# Autodesk Inventor assembly: Assembly Rack_Submission
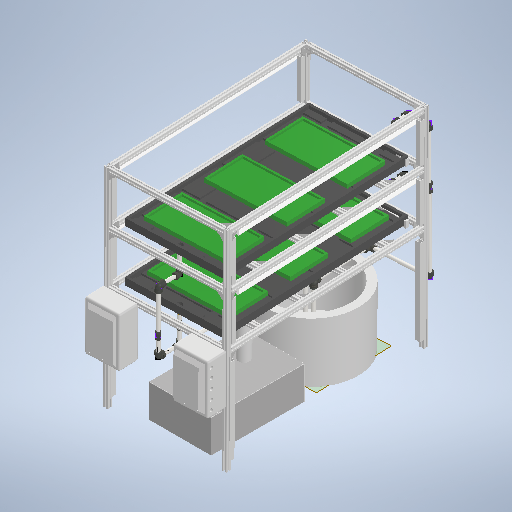
[picture p0: Inventor's stored thumbnail of the model, 512x512]
Saved by Autodesk Inventor 2025 (Build 290162000, 162)
## iProperties
Created: 2024-07-31
Part Number: Assembly Rack_Submission
Document SubType Name: Assembly
Designer: Isaac
Author: Isaac
## Documents named in this file (16)
- C:\Users\User\OneDrive\Documents\FYP\Inventor_Designs\Submission_1\Assembly Rack_Submission.iam
- C:\Users\User\OneDrive\Documents\FYP\Inventor_Designs\Submission_1\Metal_Profile 70cm.ipt
- C:\Users\User\OneDrive\Documents\FYP\Inventor_Designs\Submission_1\Light tube 118.4cm.ipt
- C:\Users\User\OneDrive\Documents\FYP\Inventor_Designs\Submission_1\flood tray.ipt
- C:\Users\User\OneDrive\Documents\FYP\Inventor_Designs\Platform\Potting Tray.ipt
- C:\Users\User\OneDrive\Documents\FYP\Inventor_Designs\Submission_1\Metal Profile 129 cm.ipt
- C:\Users\User\OneDrive\Documents\FYP\Inventor_Designs\Submission_1\Metal Profile 134 cm.ipt
- C:\Users\User\OneDrive\Documents\FYP\Inventor_Designs\L Bracket\L Angle Bracket 30x30.ipt
- C:\Users\User\OneDrive\Documents\FYP\Inventor_Designs\Submission_1\Tub.ipt
- C:\Users\User\OneDrive\Documents\FYP\Inventor_Designs\Submission_1\Water pump.ipt
- C:\Users\User\OneDrive\Documents\FYP\Inventor_Designs\Submission_1\wire box and cover.iam
- C:\Users\User\OneDrive\Documents\FYP\Inventor_Designs\Submission_1\25 cm trunk.ipt
- C:\Users\User\OneDrive\Documents\FYP\Inventor_Designs\Submission_1\55 cm trunk.ipt
- C:\Users\User\OneDrive\Documents\FYP\Inventor_Designs\Submission_1\Part245.ipt
- C:\Users\User\OneDrive\Documents\FYP\Inventor_Designs\Submission_1\Assembly Rack_Submission\AIP\Tube and Pipe\Run03\Assembly Rack_Submission.Tube and Pipe Runs.iam
- C:\Users\User\OneDrive\Documents\FYP\Inventor_Designs\Submission_1\Part18.ipt
## Components (108 placed, 15 different names)
1. Metal_Profile 70cm:1
2. Metal_Profile 70cm:2
3. Metal_Profile 70cm:3
4. Metal_Profile 70cm:4
5. Metal_Profile 70cm:5
6. Metal_Profile 70cm:6
7. Light tube 118.4cm:1
8. Light tube 118.4cm:2
9. Light tube 118.4cm:3
10. Light tube 118.4cm:4
11. flood tray:1 — Mate:196, Mate:198
12. Potting Tray:1
13. Potting Tray:2
14. Potting Tray:3
15. Potting Tray:4
16. Potting Tray:5
17. Potting Tray:6
18. Metal_Profile 70cm:7
19. Metal_Profile 70cm:8
20. flood tray:2
21. Metal Profile 129 cm:1
22. Metal Profile 129 cm:2
23. Metal Profile 129 cm:3
24. Metal Profile 129 cm:4
25. Metal Profile 134 cm:1
26. Metal Profile 134 cm:2 — Flush:117
27. Metal Profile 134 cm:3
28. Metal Profile 134 cm:4
29. Metal Profile 129 cm:5
30. Metal Profile 129 cm:6
31. Metal_Profile 70cm:9
32. Metal_Profile 70cm:10
33. Metal_Profile 70cm:11
34. Metal_Profile 70cm:12
35. Metal_Profile 70cm:13
36. Metal_Profile 70cm:14
37. L Angle Bracket 30x30:1
38. L Angle Bracket 30x30:2
39. L Angle Bracket 30x30:3
40. L Angle Bracket 30x30:4
41. L Angle Bracket 30x30:5
42. L Angle Bracket 30x30:6
43. L Angle Bracket 30x30:7
44. L Angle Bracket 30x30:8
45. L Angle Bracket 30x30:9
46. L Angle Bracket 30x30:10
47. L Angle Bracket 30x30:11
48. L Angle Bracket 30x30:12
49. L Angle Bracket 30x30:13
50. L Angle Bracket 30x30:14
51. L Angle Bracket 30x30:15
52. L Angle Bracket 30x30:16
53. L Angle Bracket 30x30:17
54. L Angle Bracket 30x30:18
55. L Angle Bracket 30x30:19
56. L Angle Bracket 30x30:20
57. L Angle Bracket 30x30:21
58. L Angle Bracket 30x30:22
59. L Angle Bracket 30x30:23
60. L Angle Bracket 30x30:24
61. L Angle Bracket 30x30:25
62. L Angle Bracket 30x30:26
63. L Angle Bracket 30x30:27
64. L Angle Bracket 30x30:28
65. L Angle Bracket 30x30:29
66. L Angle Bracket 30x30:30
67. L Angle Bracket 30x30:31
68. L Angle Bracket 30x30:32
69. L Angle Bracket 30x30:33
70. L Angle Bracket 30x30:34
71. L Angle Bracket 30x30:35
72. L Angle Bracket 30x30:36
73. L Angle Bracket 30x30:37
74. L Angle Bracket 30x30:38
75. L Angle Bracket 30x30:39
76. L Angle Bracket 30x30:40
77. L Angle Bracket 30x30:41
78. L Angle Bracket 30x30:42
79. L Angle Bracket 30x30:43
80. L Angle Bracket 30x30:44
81. L Angle Bracket 30x30:45
82. L Angle Bracket 30x30:46
83. L Angle Bracket 30x30:47
84. L Angle Bracket 30x30:48
85. L Angle Bracket 30x30:49
86. L Angle Bracket 30x30:50
87. L Angle Bracket 30x30:51
88. L Angle Bracket 30x30:52
89. Tub:1 — Mate:198, Flush:117
90. Tube & Pipe Runs [sub-assembly]
91. Water pump:1 — Mate:196, Mate:197
92. wire box and cover:1 [sub-assembly]
93. wire box and cover:2 [sub-assembly]
94. 25 cm trunk:1
95. 25 cm trunk:2
96. 25 cm trunk:3
97. 25 cm trunk:4
98. 25 cm trunk:5
99. 25 cm trunk:6
100. 25 cm trunk:7
101. 25 cm trunk:8
102. 55 cm trunk:1
103. 55 cm trunk:2
104. 55 cm trunk:3
105. 55 cm trunk:4 — Mate:197
106. Part245:1
107. Part18:3
108. Part18:4
## Relationships (315: Mate 198, Flush 117)
- [Flush] (60 mm): Metal_Profile 70cm:3 ↔ flood tray:1
- [Mate]: flood tray:1 ↔ Potting Tray:3
- [Mate]: flood tray:1 ↔ Potting Tray:1
- [Mate]: flood tray:1 ↔ Potting Tray:2
- [Mate] (30 mm): flood tray:1 ↔ Potting Tray:3
- [Mate] (50 mm): flood tray:1 ↔ Potting Tray:3
- [Mate] (30 mm): flood tray:1 ↔ Potting Tray:1
- [Mate] (150 mm): Potting Tray:1 ↔ Potting Tray:3
- [Mate] (30 mm): flood tray:1 ↔ Potting Tray:2
- [Mate] (150 mm): Potting Tray:1 ↔ Potting Tray:2
- [Mate] (150 mm): Potting Tray:4 ↔ Potting Tray:5
- [Mate] (150 mm): Potting Tray:5 ↔ Potting Tray:6
- [Mate]: Metal_Profile 70cm:8 ↔ flood tray:2
- [Flush]: flood tray:1 ↔ flood tray:2
- [Flush]: flood tray:1 ↔ flood tray:2
- [Flush]: Metal_Profile 70cm:5 ↔ Metal Profile 129 cm:3
- [Mate]: Metal_Profile 70cm:5 ↔ Metal Profile 129 cm:1
- [Flush]: Metal_Profile 70cm:5 ↔ Metal Profile 129 cm:1
- [Mate]: Metal_Profile 70cm:5 ↔ Metal Profile 134 cm:2
- [Flush]: Metal_Profile 70cm:5 ↔ Metal Profile 134 cm:2
- [Flush]: Metal Profile 129 cm:1 ↔ Metal Profile 134 cm:2
- [Flush]: Metal_Profile 70cm:5 ↔ Metal Profile 134 cm:1
- [Mate]: Metal_Profile 70cm:5 ↔ Metal Profile 134 cm:1
- [Flush]: Metal_Profile 70cm:5 ↔ Metal Profile 134 cm:1
- [Flush]: Metal_Profile 70cm:5 ↔ Metal Profile 134 cm:1
- [Flush]: Metal_Profile 70cm:5 ↔ Metal Profile 129 cm:3
- [Flush]: Metal Profile 129 cm:3 ↔ Metal Profile 134 cm:1
- [Mate]: Metal Profile 129 cm:3 ↔ Metal Profile 134 cm:1
- [Flush]: Metal Profile 129 cm:1 ↔ Metal Profile 134 cm:4
- [Mate]: Metal_Profile 70cm:6 ↔ Metal Profile 134 cm:4
- [Mate]: Metal Profile 129 cm:1 ↔ Metal Profile 134 cm:4
- [Flush]: Metal Profile 129 cm:3 ↔ Metal Profile 134 cm:3
- [Mate]: Metal Profile 129 cm:3 ↔ Metal Profile 134 cm:3
- [Mate]: Metal_Profile 70cm:6 ↔ Metal Profile 134 cm:3
- [Flush]: Metal_Profile 70cm:1 ↔ Metal Profile 129 cm:6
- [Mate]: Metal Profile 134 cm:1 ↔ Metal Profile 129 cm:6
- [Flush]: Metal Profile 134 cm:1 ↔ Metal Profile 129 cm:6
- [Mate]: Metal Profile 129 cm:4 ↔ Metal Profile 134 cm:2
- [Flush]: Metal Profile 129 cm:4 ↔ Metal Profile 134 cm:2
- [Mate]: Metal Profile 134 cm:1 ↔ Metal Profile 129 cm:5
- [Flush]: Metal Profile 134 cm:1 ↔ Metal Profile 129 cm:5
- [Mate]: Metal Profile 129 cm:2 ↔ Metal Profile 134 cm:2
- [Flush]: Metal Profile 129 cm:2 ↔ Metal Profile 134 cm:2
- [Flush]: Metal_Profile 70cm:5 ↔ Metal Profile 134 cm:2
- [Mate]: Metal_Profile 70cm:6 ↔ Metal Profile 129 cm:1
- [Flush]: Metal Profile 129 cm:3 ↔ Metal Profile 134 cm:3
- [Flush]: Metal_Profile 70cm:6 ↔ Metal Profile 134 cm:3
- [Flush] (330 mm): Metal Profile 129 cm:3 ↔ Metal Profile 129 cm:5
- [Flush] (330 mm): Metal Profile 129 cm:5 ↔ Metal Profile 129 cm:6
- [Flush] (330 mm): Metal Profile 129 cm:2 ↔ Metal Profile 129 cm:4
- [Flush]: Metal_Profile 70cm:1 ↔ Metal Profile 134 cm:2
- [Mate]: Metal_Profile 70cm:1 ↔ Metal Profile 134 cm:1
- [Flush]: Metal_Profile 70cm:3 ↔ Metal Profile 134 cm:1
- [Mate]: Metal_Profile 70cm:3 ↔ Metal Profile 134 cm:1
- [Flush]: Metal_Profile 70cm:3 ↔ Metal Profile 129 cm:2
- [Flush]: Metal_Profile 70cm:1 ↔ Metal Profile 129 cm:4
- [Flush]: Metal_Profile 70cm:2 ↔ Metal Profile 129 cm:6
- [Flush]: Metal_Profile 70cm:2 ↔ Metal Profile 134 cm:3
- [Mate]: Metal_Profile 70cm:2 ↔ Metal Profile 134 cm:3
- [Flush]: Metal_Profile 70cm:4 ↔ Metal Profile 129 cm:5
- [Flush]: Metal_Profile 70cm:4 ↔ Metal Profile 134 cm:3
- [Mate]: Metal_Profile 70cm:4 ↔ Metal Profile 134 cm:3
- [Flush]: Light tube 118.4cm:3 ↔ Metal Profile 129 cm:3
- [Mate] (50 mm): Light tube 118.4cm:3 ↔ Metal Profile 134 cm:1
- [Mate]: Light tube 118.4cm:3 ↔ Metal Profile 129 cm:3
- [Mate]: Light tube 118.4cm:2 ↔ Metal Profile 129 cm:5
- [Flush]: Light tube 118.4cm:2 ↔ Metal Profile 129 cm:5
- [Mate] (50 mm): Light tube 118.4cm:2 ↔ Metal Profile 134 cm:1
- [Flush]: Light tube 118.4cm:1 ↔ Metal Profile 129 cm:1
- [Mate] (50 mm): Light tube 118.4cm:1 ↔ Metal Profile 134 cm:2
- [Mate]: Light tube 118.4cm:1 ↔ Metal Profile 129 cm:1
- [Mate] (50 mm): Light tube 118.4cm:4 ↔ Metal Profile 134 cm:2
- [Flush]: Light tube 118.4cm:4 ↔ Metal Profile 129 cm:2
- [Mate]: Light tube 118.4cm:4 ↔ Metal Profile 129 cm:2
- [Mate]: Metal_Profile 70cm:7 ↔ Metal Profile 129 cm:6
- [Flush]: Metal_Profile 70cm:7 ↔ Metal Profile 129 cm:6
- [Mate] (200 mm): Metal_Profile 70cm:1 ↔ Metal_Profile 70cm:7
- [Flush]: Metal_Profile 70cm:8 ↔ Metal Profile 129 cm:6
- [Mate]: Metal_Profile 70cm:8 ↔ Metal Profile 129 cm:6
- [Mate] (200 mm): Metal_Profile 70cm:2 ↔ Metal_Profile 70cm:8
- [Mate]: Metal Profile 129 cm:6 ↔ Metal_Profile 70cm:12
- [Flush]: Metal Profile 129 cm:6 ↔ Metal_Profile 70cm:12
- [Mate] (255 mm): Metal_Profile 70cm:7 ↔ Metal_Profile 70cm:12
- [Mate]: Metal Profile 129 cm:6 ↔ Metal_Profile 70cm:11
- [Flush]: Metal Profile 129 cm:6 ↔ Metal_Profile 70cm:11
- [Mate] (255 mm): Metal_Profile 70cm:8 ↔ Metal_Profile 70cm:11
- [Mate]: Metal Profile 129 cm:5 ↔ Metal_Profile 70cm:10
- [Flush]: Metal Profile 129 cm:5 ↔ Metal_Profile 70cm:10
- [Mate] (200 mm): Metal_Profile 70cm:3 ↔ Metal_Profile 70cm:10
- [Mate]: Metal Profile 129 cm:5 ↔ Metal_Profile 70cm:9
- [Flush]: Metal Profile 129 cm:5 ↔ Metal_Profile 70cm:9
- [Mate] (255 mm): Metal_Profile 70cm:9 ↔ Metal_Profile 70cm:10
- [Mate]: Metal Profile 129 cm:5 ↔ Metal_Profile 70cm:14
- [Flush]: Metal Profile 129 cm:5 ↔ Metal_Profile 70cm:14
- [Mate] (200 mm): Metal_Profile 70cm:4 ↔ Metal_Profile 70cm:14
- [Mate]: Metal Profile 129 cm:5 ↔ Metal_Profile 70cm:13
- [Flush]: Metal Profile 129 cm:5 ↔ Metal_Profile 70cm:13
- [Mate] (255 mm): Metal_Profile 70cm:13 ↔ Metal_Profile 70cm:14
- [Mate]: Metal_Profile 70cm:7 ↔ flood tray:2
- [Flush] (75 mm): flood tray:2 ↔ Metal Profile 129 cm:6
- [Mate]: flood tray:1 ↔ Metal_Profile 70cm:9
- [Flush]: Metal Profile 129 cm:1 ↔ L Angle Bracket 30x30:1
- [Mate]: Metal_Profile 70cm:5 ↔ L Angle Bracket 30x30:1
- [Mate]: Metal Profile 129 cm:1 ↔ L Angle Bracket 30x30:1
- [Mate]: Metal Profile 129 cm:1 ↔ L Angle Bracket 30x30:6
- [Flush]: Metal Profile 129 cm:1 ↔ L Angle Bracket 30x30:6
- [Mate]: Metal_Profile 70cm:6 ↔ L Angle Bracket 30x30:6
- [Flush]: Metal Profile 129 cm:2 ↔ L Angle Bracket 30x30:5
- [Mate]: Metal_Profile 70cm:4 ↔ L Angle Bracket 30x30:4
- [Flush]: Metal_Profile 70cm:4 ↔ L Angle Bracket 30x30:4
- [Mate]: Metal Profile 129 cm:2 ↔ L Angle Bracket 30x30:4
- [Mate]: Metal Profile 129 cm:2 ↔ L Angle Bracket 30x30:5
- [Flush]: Metal Profile 129 cm:2 ↔ L Angle Bracket 30x30:5
- [Mate]: Metal_Profile 70cm:14 ↔ L Angle Bracket 30x30:5
- [Flush]: Metal Profile 129 cm:2 ↔ L Angle Bracket 30x30:7
- [Mate]: Metal_Profile 70cm:13 ↔ L Angle Bracket 30x30:2
- [Mate]: Metal Profile 129 cm:2 ↔ L Angle Bracket 30x30:2
- [Flush]: Metal Profile 129 cm:2 ↔ L Angle Bracket 30x30:2
- [Flush]: Metal Profile 129 cm:2 ↔ L Angle Bracket 30x30:7
- [Mate]: Metal_Profile 70cm:9 ↔ L Angle Bracket 30x30:7
- [Mate]: Metal Profile 129 cm:2 ↔ L Angle Bracket 30x30:7
- [Mate]: Metal_Profile 70cm:10 ↔ L Angle Bracket 30x30:3
- [Flush]: Metal_Profile 70cm:10 ↔ L Angle Bracket 30x30:3
- [Mate]: Metal Profile 129 cm:2 ↔ L Angle Bracket 30x30:3
- [Flush]: Metal Profile 129 cm:4 ↔ L Angle Bracket 30x30:10
- [Mate]: Metal Profile 129 cm:4 ↔ L Angle Bracket 30x30:10
- [Mate]: Metal_Profile 70cm:2 ↔ L Angle Bracket 30x30:10
- [Mate]: Metal_Profile 70cm:8 ↔ L Angle Bracket 30x30:12
- [Mate]: Metal Profile 129 cm:4 ↔ L Angle Bracket 30x30:12
- [Flush]: Metal Profile 129 cm:4 ↔ L Angle Bracket 30x30:12
- [Mate]: Metal_Profile 70cm:11 ↔ L Angle Bracket 30x30:8
- [Flush]: Metal_Profile 70cm:11 ↔ L Angle Bracket 30x30:8
- [Mate]: Metal Profile 129 cm:4 ↔ L Angle Bracket 30x30:8
- [Flush]: Metal_Profile 70cm:12 ↔ L Angle Bracket 30x30:11
- [Mate]: Metal Profile 129 cm:4 ↔ L Angle Bracket 30x30:11
- [Mate]: Metal_Profile 70cm:12 ↔ L Angle Bracket 30x30:11
- [Flush]: Metal Profile 129 cm:4 ↔ L Angle Bracket 30x30:11
- [Mate]: Metal_Profile 70cm:7 ↔ L Angle Bracket 30x30:9
- [Flush]: Metal_Profile 70cm:7 ↔ L Angle Bracket 30x30:9
- [Mate]: Metal Profile 129 cm:4 ↔ L Angle Bracket 30x30:9
- [Mate]: Metal_Profile 70cm:3 ↔ L Angle Bracket 30x30:13
- [Mate]: Metal Profile 129 cm:2 ↔ L Angle Bracket 30x30:13
- [Flush]: Metal_Profile 70cm:1 ↔ L Angle Bracket 30x30:14
- [Mate]: Metal_Profile 70cm:1 ↔ L Angle Bracket 30x30:14
- [Flush]: Metal_Profile 70cm:1 ↔ L Angle Bracket 30x30:14
- [Mate]: Metal Profile 129 cm:4 ↔ L Angle Bracket 30x30:14
- [Mate]: Metal_Profile 70cm:5 ↔ L Angle Bracket 30x30:15
- [Flush]: Metal Profile 134 cm:2 ↔ L Angle Bracket 30x30:15
- [Mate]: Metal Profile 134 cm:2 ↔ L Angle Bracket 30x30:15
- [Mate]: Metal_Profile 70cm:3 ↔ L Angle Bracket 30x30:16
- [Flush]: Metal Profile 134 cm:2 ↔ L Angle Bracket 30x30:16
- [Mate]: Metal Profile 134 cm:2 ↔ L Angle Bracket 30x30:16
- [Mate]: Metal_Profile 70cm:1 ↔ L Angle Bracket 30x30:26
- [Flush]: Metal_Profile 70cm:1 ↔ L Angle Bracket 30x30:26
- [Mate]: Metal Profile 134 cm:2 ↔ L Angle Bracket 30x30:26
- [Mate]: Metal_Profile 70cm:6 ↔ L Angle Bracket 30x30:23
- [Flush]: Metal_Profile 70cm:6 ↔ L Angle Bracket 30x30:23
- [Mate]: Metal Profile 134 cm:4 ↔ L Angle Bracket 30x30:23
- [Mate]: Metal_Profile 70cm:4 ↔ L Angle Bracket 30x30:19
- [Flush]: Metal Profile 134 cm:4 ↔ L Angle Bracket 30x30:19
- [Mate]: Metal Profile 134 cm:4 ↔ L Angle Bracket 30x30:19
- [Mate]: Metal_Profile 70cm:2 ↔ L Angle Bracket 30x30:22
- [Flush]: Metal Profile 134 cm:4 ↔ L Angle Bracket 30x30:22
- [Mate]: Metal Profile 134 cm:4 ↔ L Angle Bracket 30x30:22
- [Mate]: Metal_Profile 70cm:5 ↔ L Angle Bracket 30x30:24
- [Flush]: Metal Profile 134 cm:1 ↔ L Angle Bracket 30x30:24
- [Mate]: Metal Profile 134 cm:1 ↔ L Angle Bracket 30x30:24
- [Mate]: Metal_Profile 70cm:3 ↔ L Angle Bracket 30x30:17
- [Flush]: Metal Profile 134 cm:1 ↔ L Angle Bracket 30x30:17
- [Mate]: Metal Profile 134 cm:1 ↔ L Angle Bracket 30x30:17
- [Mate]: Metal_Profile 70cm:1 ↔ L Angle Bracket 30x30:25
- [Flush]: Metal Profile 134 cm:1 ↔ L Angle Bracket 30x30:25
- [Mate]: Metal Profile 134 cm:1 ↔ L Angle Bracket 30x30:25
- [Mate]: Metal Profile 129 cm:3 ↔ L Angle Bracket 30x30:18
- [Flush]: Metal Profile 134 cm:1 ↔ L Angle Bracket 30x30:18
- [Mate]: Metal Profile 134 cm:1 ↔ L Angle Bracket 30x30:18
- [Flush]: Metal Profile 134 cm:1 ↔ L Angle Bracket 30x30:21
- [Mate]: Metal Profile 129 cm:5 ↔ L Angle Bracket 30x30:21
- [Mate]: Metal Profile 134 cm:1 ↔ L Angle Bracket 30x30:21
- [Flush]: Metal Profile 134 cm:1 ↔ L Angle Bracket 30x30:20
- [Mate]: Metal Profile 134 cm:1 ↔ L Angle Bracket 30x30:20
- [Mate]: Metal Profile 129 cm:6 ↔ L Angle Bracket 30x30:20
- [Flush]: Metal Profile 134 cm:3 ↔ L Angle Bracket 30x30:29
- [Mate]: Metal Profile 129 cm:6 ↔ L Angle Bracket 30x30:29
- [Mate]: Metal Profile 134 cm:3 ↔ L Angle Bracket 30x30:29
- [Flush]: Metal Profile 134 cm:3 ↔ L Angle Bracket 30x30:28
- [Mate]: Metal Profile 129 cm:5 ↔ L Angle Bracket 30x30:28
- [Mate]: Metal Profile 134 cm:3 ↔ L Angle Bracket 30x30:28
- [Mate]: Metal Profile 129 cm:3 ↔ L Angle Bracket 30x30:27
- [Flush]: Metal Profile 129 cm:3 ↔ L Angle Bracket 30x30:27
- [Mate]: Metal Profile 134 cm:3 ↔ L Angle Bracket 30x30:27
- [Mate]: Metal Profile 129 cm:4 ↔ L Angle Bracket 30x30:30
- [Flush]: Metal Profile 129 cm:4 ↔ L Angle Bracket 30x30:30
- [Mate]: Metal Profile 134 cm:4 ↔ L Angle Bracket 30x30:30
- [Mate]: Metal Profile 129 cm:2 ↔ L Angle Bracket 30x30:31
- [Flush]: Metal Profile 129 cm:2 ↔ L Angle Bracket 30x30:31
- [Mate]: Metal Profile 134 cm:4 ↔ L Angle Bracket 30x30:31
- [Mate]: Metal Profile 129 cm:1 ↔ L Angle Bracket 30x30:32
- [Flush]: Metal Profile 129 cm:1 ↔ L Angle Bracket 30x30:32
- [Mate]: Metal Profile 134 cm:4 ↔ L Angle Bracket 30x30:32
- [Mate]: Metal Profile 129 cm:1 ↔ L Angle Bracket 30x30:34
- [Mate]: Metal Profile 134 cm:2 ↔ L Angle Bracket 30x30:34
- [Flush]: Metal Profile 129 cm:1 ↔ L Angle Bracket 30x30:34
- [Mate]: Metal Profile 129 cm:2 ↔ L Angle Bracket 30x30:35
- [Mate]: Metal Profile 134 cm:2 ↔ L Angle Bracket 30x30:35
- [Flush]: Metal Profile 129 cm:2 ↔ L Angle Bracket 30x30:35
- [Mate]: Metal Profile 129 cm:4 ↔ L Angle Bracket 30x30:33
- [Mate]: Metal Profile 134 cm:2 ↔ L Angle Bracket 30x30:33
- [Flush]: Metal Profile 129 cm:4 ↔ L Angle Bracket 30x30:33
- [Mate]: Metal_Profile 70cm:6 ↔ L Angle Bracket 30x30:36
- [Flush]: Metal_Profile 70cm:6 ↔ L Angle Bracket 30x30:36
- [Mate]: Metal Profile 134 cm:3 ↔ L Angle Bracket 30x30:36
- [Mate]: Metal_Profile 70cm:4 ↔ L Angle Bracket 30x30:37
- [Mate]: Metal Profile 134 cm:3 ↔ L Angle Bracket 30x30:37
- [Flush]: Metal_Profile 70cm:4 ↔ L Angle Bracket 30x30:37
- [Mate]: Metal_Profile 70cm:2 ↔ L Angle Bracket 30x30:38
- [Flush]: Metal_Profile 70cm:2 ↔ L Angle Bracket 30x30:38
- [Mate]: Metal Profile 134 cm:3 ↔ L Angle Bracket 30x30:38
- [Flush]: Metal_Profile 70cm:5 ↔ L Angle Bracket 30x30:40
- [Mate]: Metal Profile 129 cm:3 ↔ L Angle Bracket 30x30:40
- [Mate]: Metal_Profile 70cm:5 ↔ L Angle Bracket 30x30:40
- [Flush]: Metal_Profile 70cm:5 ↔ L Angle Bracket 30x30:40
- [Flush]: Metal_Profile 70cm:3 ↔ L Angle Bracket 30x30:39
- [Mate]: Metal Profile 129 cm:5 ↔ L Angle Bracket 30x30:39
- [Mate]: Metal_Profile 70cm:3 ↔ L Angle Bracket 30x30:39
- [Flush]: Metal_Profile 70cm:1 ↔ L Angle Bracket 30x30:41
- [Mate]: Metal Profile 129 cm:6 ↔ L Angle Bracket 30x30:41
- [Mate]: Metal_Profile 70cm:1 ↔ L Angle Bracket 30x30:41
- [Flush]: Metal_Profile 70cm:10 ↔ L Angle Bracket 30x30:45
- [Mate]: Metal Profile 129 cm:5 ↔ L Angle Bracket 30x30:45
- [Mate]: Metal_Profile 70cm:10 ↔ L Angle Bracket 30x30:45
- [Flush]: Metal_Profile 70cm:9 ↔ L Angle Bracket 30x30:49
- [Mate]: Metal Profile 129 cm:5 ↔ L Angle Bracket 30x30:48
- [Mate]: Metal_Profile 70cm:9 ↔ L Angle Bracket 30x30:48
- [Flush]: Metal_Profile 70cm:9 ↔ L Angle Bracket 30x30:48
- [Flush]: Metal_Profile 70cm:13 ↔ L Angle Bracket 30x30:49
- [Mate]: Metal Profile 129 cm:5 ↔ L Angle Bracket 30x30:49
- [Mate]: Metal_Profile 70cm:13 ↔ L Angle Bracket 30x30:49
- [Flush]: Metal_Profile 70cm:14 ↔ L Angle Bracket 30x30:43
- [Mate]: Metal Profile 129 cm:5 ↔ L Angle Bracket 30x30:43
- [Mate]: Metal_Profile 70cm:14 ↔ L Angle Bracket 30x30:43
- [Flush]: Metal_Profile 70cm:7 ↔ L Angle Bracket 30x30:44
- [Mate]: Metal Profile 129 cm:6 ↔ L Angle Bracket 30x30:44
- [Mate]: Metal_Profile 70cm:7 ↔ L Angle Bracket 30x30:44
- [Flush]: Metal_Profile 70cm:12 ↔ L Angle Bracket 30x30:42
- [Mate]: Metal Profile 129 cm:6 ↔ L Angle Bracket 30x30:42
- [Mate]: Metal_Profile 70cm:12 ↔ L Angle Bracket 30x30:42
- [Mate]: Metal Profile 129 cm:6 ↔ L Angle Bracket 30x30:47
- [Flush]: Metal Profile 129 cm:6 ↔ L Angle Bracket 30x30:47
- [Mate]: Metal_Profile 70cm:11 ↔ L Angle Bracket 30x30:47
- [Flush]: Metal_Profile 70cm:8 ↔ L Angle Bracket 30x30:46
- [Mate]: Metal Profile 129 cm:6 ↔ L Angle Bracket 30x30:46
- [Mate]: Metal_Profile 70cm:8 ↔ L Angle Bracket 30x30:46
- [Mate]: Metal Profile 129 cm:3 ↔ L Angle Bracket 30x30:51
- [Flush]: Metal Profile 129 cm:3 ↔ L Angle Bracket 30x30:51
- [Mate]: Metal_Profile 70cm:6 ↔ L Angle Bracket 30x30:51
- [Flush]: Metal Profile 129 cm:5 ↔ L Angle Bracket 30x30:50
- [Mate]: Metal_Profile 70cm:4 ↔ L Angle Bracket 30x30:50
- [Mate]: Metal Profile 129 cm:5 ↔ L Angle Bracket 30x30:50
- [Mate]: Metal Profile 129 cm:6 ↔ L Angle Bracket 30x30:52
- [Flush]: Metal Profile 129 cm:6 ↔ L Angle Bracket 30x30:52
- [Mate]: Metal_Profile 70cm:2 ↔ L Angle Bracket 30x30:52
- [Mate]: Metal_Profile 70cm:1 ↔ wire box and cover:2
- [Flush]: Metal_Profile 70cm:1 ↔ wire box and cover:2
- [Flush]: Metal Profile 134 cm:2 ↔ wire box and cover:2
- [Mate]: Metal Profile 134 cm:1 ↔ wire box and cover:1
- [Flush]: Metal_Profile 70cm:1 ↔ wire box and cover:1
- [Flush]: Metal Profile 134 cm:1 ↔ wire box and cover:1
- [Mate]: Metal Profile 134 cm:2 ↔ 25 cm trunk:1
- [Flush]: Metal Profile 134 cm:2 ↔ 25 cm trunk:1
- [Mate] (20 mm): Metal Profile 129 cm:4 ↔ 25 cm trunk:1
- [Mate]: Metal Profile 134 cm:2 ↔ 25 cm trunk:4
- [Flush]: Metal Profile 134 cm:2 ↔ 25 cm trunk:4
- [Mate] (20 mm): Metal Profile 129 cm:2 ↔ 25 cm trunk:4
- [Mate]: Metal Profile 134 cm:1 ↔ 25 cm trunk:2
- [Flush]: Metal Profile 134 cm:1 ↔ 25 cm trunk:2
- [Mate] (20 mm): Metal Profile 129 cm:6 ↔ 25 cm trunk:2
- [Mate]: Metal Profile 134 cm:1 ↔ 25 cm trunk:7
- [Flush]: Metal Profile 134 cm:1 ↔ 25 cm trunk:7
- [Mate] (20 mm): Metal Profile 129 cm:2 ↔ 25 cm trunk:7
- [Mate]: Metal Profile 134 cm:4 ↔ 25 cm trunk:3
- [Flush]: Metal Profile 134 cm:4 ↔ 25 cm trunk:3
- [Mate] (20 mm): Metal Profile 129 cm:4 ↔ 25 cm trunk:3
- [Mate]: Metal Profile 134 cm:3 ↔ 25 cm trunk:8
- [Flush]: Metal Profile 134 cm:3 ↔ 25 cm trunk:8
- [Mate] (20 mm): Metal Profile 129 cm:4 ↔ 25 cm trunk:8
- [Mate]: Metal Profile 134 cm:3 ↔ 25 cm trunk:5
- [Flush]: Metal Profile 134 cm:3 ↔ 25 cm trunk:5
- [Mate] (20 mm): Metal Profile 129 cm:5 ↔ 25 cm trunk:5
- [Mate]: Metal Profile 134 cm:4 ↔ 25 cm trunk:6
- [Flush]: Metal Profile 134 cm:4 ↔ 25 cm trunk:6
- [Mate] (20 mm): Metal Profile 129 cm:2 ↔ 25 cm trunk:6
- [Mate]: Metal Profile 134 cm:2 ↔ 55 cm trunk:3
- [Flush]: Metal Profile 134 cm:2 ↔ 55 cm trunk:3
- [Mate] (50 mm): Metal Profile 129 cm:4 ↔ 55 cm trunk:3
- [Mate]: Metal Profile 134 cm:4 ↔ 55 cm trunk:4
- [Mate]: Metal Profile 134 cm:4 ↔ 55 cm trunk:4
- [Mate] (50 mm): Metal Profile 129 cm:4 ↔ 55 cm trunk:4
- [Mate]: Metal Profile 134 cm:1 ↔ 55 cm trunk:2
- [Mate]: Metal Profile 134 cm:1 ↔ 55 cm trunk:2
- [Mate] (50 mm): Metal Profile 129 cm:6 ↔ 55 cm trunk:2
- [Mate]: Metal Profile 134 cm:3 ↔ 55 cm trunk:1
- [Mate]: Metal Profile 134 cm:3 ↔ 55 cm trunk:1
- [Mate] (50 mm): Metal Profile 129 cm:6 ↔ 55 cm trunk:1
- [Mate]: Potting Tray:6 ↔ flood tray:2
- [Mate] (30 mm): Potting Tray:6 ↔ flood tray:2
- [Mate] (50 mm): Potting Tray:6 ↔ flood tray:2
- [Mate]: Potting Tray:5 ↔ flood tray:2
- [Mate] (30 mm): Potting Tray:5 ↔ flood tray:2
- [Mate]: Potting Tray:4 ↔ flood tray:2
- [Mate] (30 mm): Potting Tray:4 ↔ flood tray:2
- Mate:196 (520 mm): flood tray:1 ↔ Water pump:1
- Mate:197 (730 mm): Water pump:1 ↔ 55 cm trunk:4
- Mate:198 (630 mm): flood tray:1 ↔ Tub:1
- Flush:117: Metal Profile 134 cm:2 ↔ Tub:1
## Named parameters: d0_d171 = 0 mm, d1_d172 = 0 mm, d2_d173 = 0 mm, d16_d98 = 60 mm, d103_d113 = 150 mm, d104_d114 = 30 mm, d105_d115 = 150 mm, d109_d119 = 150 mm, d8_d104 = 0 mm, d143_d304 = 0 mm, d144_d305 = 0 mm, d145_d306 = 0 mm, d146_d307 = 0 mm, d147_d308 = 0 mm, d148_d309 = 0 mm, d149_d310 = 0 mm, d150_d311 = 0 mm, d151_d312 = 0 mm, d152_d313 = 0 mm, d153_d314 = 0 mm, d176_d272 = 0 mm, d177_d273 = 0 mm, d178_d274 = 0 mm, d179_d276 = 0 mm, d180_d277 = 0 mm, d181_d278 = 0 mm, d182_d279 = 0 mm, d183_d280 = 0 mm, d184_d281 = 0 mm, d185_d282 = 0 mm, d186_d283 = 0 mm, d187_d284 = 0 mm, d188_d285 = 0 mm, d189_d286 = 0 mm, d190_d287 = 0 mm, d191_d288 = 0 mm, d192_d289 = 0 mm, d193_d290 = 0 mm, d194_d291 = 0 mm, d195_d292 = 0 mm, d196_d293 = 0 mm, d197_d294 = 0 mm, d198_d296 = 0 mm, d199_d297 = 0 mm, d200_d298 = 0 mm, d201_d299 = 0 mm, d202_d300 = 0 mm, d203_d301 = 0 mm, d204_d302 = 0 mm, d205_d303 = 0 mm, d206_d238 = 200 mm, d207_d239 = 0 mm, d208_d240 = 0 mm, d209_d241 = 255 mm, d210_d242 = 0 mm, d211_d243 = 0 mm, d212_d244 = 200 mm, d213_d245 = 0 mm, d214_d246 = 0 mm, d215_d247 = 255 mm, d216_d248 = 0 mm, d217_d249 = 75 mm, d218_d250 = 0 mm, d219_d254 = 0 mm, d220_d255 = 0 mm, d221_d256 = 0 mm, d222_d258 = 0 mm, d223_d259 = 0 mm, d224_d260 = 0 mm, d225_d261 = 0 mm, d226_d262 = 0 mm, d227_d263 = 0 mm, d228_d264 = 0 mm, d229_d265 = 0 mm, d230_d266 = 0 mm, d231_d267 = 0 mm, d232_d268 = 0 mm, d233_d269 = 0 mm, d234_d270 = 0 mm, d235_d271 = 0 mm
